# Autodesk Inventor assembly: BuddyRobotASM
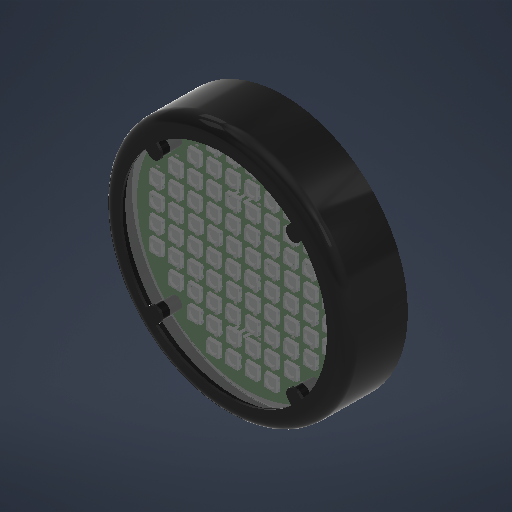
[picture p0: Inventor's stored thumbnail of the model, 512x512]
Saved by Autodesk Inventor 2026.2 (Build 302298000, 298)
## iProperties
Created: 2026-06-05
Part Number: BuddyRobotASM
Document SubType Name: Assembly
Designer: User
Author: User
## Documents named in this file (5)
- C:\Users\User\MyWorkspaces\DesktopBuddyRobot\BuddyRobot3DModel\BuddyRobotASM.iam
- C:\Users\User\MyWorkspaces\DesktopBuddyRobot\BuddyRobot3DModel\DisplayCover.ipt
- C:\Users\User\MyWorkspaces\DesktopBuddyRobot\BuddyRobot3DModel\DisplayGlassDark.ipt
- C:\Users\User\MyWorkspaces\DesktopBuddyRobot\BuddyRobot3DModel\DisplayGlass.ipt
- C:\Users\User\MyWorkspaces\DesktopBuddyRobot\BuddyRobot3DModel\Display\Display\Display.iam
## Components (4 placed, 4 different names)
1. DisplayCover:1 — Mate:1, Insert:1, Insert:2, Mate:4, Mate:5, Insert:3, Insert:4
2. DisplayGlassDark:1 — Mate:1, Insert:1, Insert:2, Mate:2, Mate:3
3. DisplayGlass:1 — Mate:2, Mate:3, Mate:4
4. Display:1 [sub-assembly] — Mate:5, Insert:3, Insert:4
## Relationships (9: Mate 5, Insert 4)
- Mate:1: DisplayCover:1 ↔ DisplayGlassDark:1
- Insert:1: DisplayCover:1 ↔ DisplayGlassDark:1
- Insert:2: DisplayCover:1 ↔ DisplayGlassDark:1
- Mate:2: DisplayGlassDark:1 ↔ DisplayGlass:1
- Mate:3: DisplayGlassDark:1 ↔ DisplayGlass:1
- Mate:4: DisplayCover:1 ↔ DisplayGlass:1
- Mate:5: DisplayCover:1 ↔ Display:1
- Insert:3: DisplayCover:1 ↔ Display:1
- Insert:4: DisplayCover:1 ↔ Display:1
